# Autodesk Inventor assembly: HBLFSN5-SEC
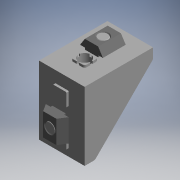
[picture p0: Inventor's stored thumbnail of the model, 180x180]
Saved by Autodesk Inventor 2017.3 (Build 213256000, 256)
## iProperties
Category: PARTsolutions
Company: MISUMI
Part Number: HBLFSN5-SEC
Catalog Web Link: www.cadenas.de
Description: HBLFSN5, HBLFSN5-4, HBLFSNB5, HBLFSNM5, HBLFSNK5, HBLFSNE5-Brackets HFS5 Reversal Brackets with Tab
Vendor: MISUMI
Document SubType Name: Assembly
Designer: partserver
Manufacturer: MISUMI
Mass: 7.80989 g
Surface Area: 64.8523 cm^2
Volume: 7.80989 cm^3
Density: 1 g/cm^3
Title: HBLFSN5-SEC
Author: Cadenas PARTsolutions
Comments: Brackets HFS5 Reversal Brackets with Tab
PSOL_IDENT_0: {$CADENAS_DATA\23d-libs\misumi\metric\38_al_extrusions_blackets\5\hblfsnm5_asmtab.prj},228 {VTYP=3D}
PSOL_IDENT_1: ,{STYP=ASSTAB},{NB=HBLFSN5-SEC},{LINA=HBLFSN5-SEC},{NN=HBLFSN5, HBLFSN5-4, HBLFSNB5, HBLFSNM5, HBLFS
PSOL_IDENT_2: NK5, HBLFSNE5},{DATE=09.09.2019 15:28:10},{GEOMDATE=14.12.2010},{VERSION=},{LINEID=10},{WBVAR=ALT1,A
PSOL_IDENT_3: LT2},{WBNUMERIC=}  {NB=HBLFSN5-SEC},{LINA=HBLFSN5-SEC},{KT=1},{PN=HBLFSN5-SEC},{TP=HBLFSN5},{NOH=1},
PSOL_IDENT_4: {NOHV=2},{MAT=ADC12},{ST=-},{TYPE=HBLFSN5},{FEAT=Reversal Bracket with Tab},{ALT1=},{ALT2=-SEC},{MAS
PSOL_IDENT_5: S=15},{AB=HCBST5-12},{NOB=2},{AN=HNTT5-5},{NON=2},{AL=1176},{W=20},{H=30},{DP=30},{T=5.0},{HDIS=8},{
PSOL_IDENT_6: DPOS=12},{HH1=18},{HV1=10},{DIA=5.3},{ALT1ALG='','w/o C (Mounting Holes for Cover)','-C','with C (Mo
PSOL_IDENT_7: unting Holes for Cover)'},{ALT2ALG= '' , 'w/o Set Applicable Bolt & Nut' , '-SET' , 'with SET (Set A
PSOL_IDENT_8: pplicable Bolt & Nut)' , '-SST' , 'with SST (Stainless Steel Set Applicable Bolt & Nut)' , '-SEU' , '
PSOL_IDENT_9: with SEU (Pre-Assy. Insertion Spring Nuts Set Applicable Bolt & Nut)' , '-SSU' , 'with SSU (Pre-Assy
PSOL_IDENT_10: . Insertion Spring Nuts Stainless Steel Set Applicable Bolt & Nut)' , '-SEP' , 'with SEP (Post-Assy.
PSOL_IDENT_11: Insertion Spring Nuts Set Applicable Bolt & Nut)' , '-SSP' , 'with SSP (Post-Assy. Insertion Spring
PSOL_IDENT_12: Nuts Set Applicable Bolt & Nut)' , '-SEC' , 'with SEC (Captured Washer Screws Nuts)' },{R=1},{R1=0.
PSOL_IDENT_13: 3},{APOSV=0},{VER=1},{PR=1},{TT=1.0},{T1=1},{TIP=HBLFSN5},{PPATH=hblfsl5_asmtpl.prj},{ABT=HCBST5-},{
PSOL_IDENT_14: ABL=12}
NB: HBLFSN5-SEC
NN: HBLFSN5, HBLFSN5-4, HBLFSNB5, HBLFSNM5, HBLFSNK5, HBLFSNE5
NT: Brackets HFS5 Reversal Brackets with Tab
NBSYN: $PN.
LINA: HBLFSN5-SEC
CATALOG: Misumi
PN: HBLFSN5-SEC
TP: HBLFSN5
MAT: ADC12
ST: -
FEAT: Reversal Bracket with Tab
ALT1: w/o C (Mounting Holes for Cover)
ALT2: with SEC (Captured Washer Screws Nuts)
MASS: 15
AB: HCBST5-12
NOB: 2
AN: HNTT5-5
NON: 2
AL: 1176
SUPPLIER: MISUMI
ARTICLENO: HBLFSN5-SEC
BOMINFO: HBLFSN5-SEC
CREATOR: CADENAS GmbH
## Documents named in this file (6)
- e:\temp\worker_16\temp\exporttempdir_9944_28_AWgfp\format_0\HBLFSN5-SEC.iam
- e:\temp\worker_16\temp\exporttempdir_9944_28_AWgfp\format_0\HBLFSN5-SECh5.ipt
- e:\temp\worker_16\temp\exporttempdir_9944_28_AWgfp\format_0\HCBST5-12_Screw.ipt
- e:\temp\worker_16\temp\exporttempdir_9944_28_AWgfp\format_0\HCBST5_w1.ipt
- e:\temp\worker_16\temp\exporttempdir_9944_28_AWgfp\format_0\SPWF5.ipt
- e:\temp\worker_16\temp\exporttempdir_9944_28_AWgfp\format_0\HNTT5-5_1.ipt
## Components (9 placed, 5 different names)
1. HBLFSN5-SECh5:1 — to_bolt_row_4_to_7_Z@1 <-> screw_to_body_Z@2, to_bolt_row_4_to_7_Z@1 <-> spring_washer_to_bolt_Z@3, to_bolt_row_4_to_7_Z@1 <-> plain_washer_to_bolt_Z@4, to_bolt_row_4_to_7_Z@1 <-> to_frames_Z@5, to_bolt_4_7_base_Z@1 <-> screw_to_body_Z@6, to_bolt_4_7_base_Z@1 <-> spring_washer_to_bolt_Z@7, to_bolt_4_7_base_Z@1 <-> plain_washer_to_bolt_Z@8, to_bolt_4_7_base_Z@1 <-> to_frames_Z@9
2. HCBST5-12_Screw:1 — to_bolt_row_4_to_7_Z@1 <-> screw_to_body_Z@2
3. HCBST5_w1:1 — to_bolt_row_4_to_7_Z@1 <-> spring_washer_to_bolt_Z@3
4. SPWF5:1 — to_bolt_row_4_to_7_Z@1 <-> plain_washer_to_bolt_Z@4
5. HNTT5-5_1:1 — to_bolt_row_4_to_7_Z@1 <-> to_frames_Z@5
6. HCBST5-12_Screw:2 — to_bolt_4_7_base_Z@1 <-> screw_to_body_Z@6
7. HCBST5_w1:2 — to_bolt_4_7_base_Z@1 <-> spring_washer_to_bolt_Z@7
8. SPWF5:2 — to_bolt_4_7_base_Z@1 <-> plain_washer_to_bolt_Z@8
9. HNTT5-5_1:2 — to_bolt_4_7_base_Z@1 <-> to_frames_Z@9
## Relationships (8: Mate 8)
- to_bolt_row_4_to_7_Z@1 <-> screw_to_body_Z@2 [Mate]: HBLFSN5-SECh5:1 ↔ HCBST5-12_Screw:1
- to_bolt_row_4_to_7_Z@1 <-> spring_washer_to_bolt_Z@3 [Mate]: HBLFSN5-SECh5:1 ↔ HCBST5_w1:1
- to_bolt_row_4_to_7_Z@1 <-> plain_washer_to_bolt_Z@4 [Mate]: HBLFSN5-SECh5:1 ↔ SPWF5:1
- to_bolt_row_4_to_7_Z@1 <-> to_frames_Z@5 [Mate]: HBLFSN5-SECh5:1 ↔ HNTT5-5_1:1
- to_bolt_4_7_base_Z@1 <-> screw_to_body_Z@6 [Mate]: HBLFSN5-SECh5:1 ↔ HCBST5-12_Screw:2
- to_bolt_4_7_base_Z@1 <-> spring_washer_to_bolt_Z@7 [Mate]: HBLFSN5-SECh5:1 ↔ HCBST5_w1:2
- to_bolt_4_7_base_Z@1 <-> plain_washer_to_bolt_Z@8 [Mate]: HBLFSN5-SECh5:1 ↔ SPWF5:2
- to_bolt_4_7_base_Z@1 <-> to_frames_Z@9 [Mate]: HBLFSN5-SECh5:1 ↔ HNTT5-5_1:2
